# Autodesk Inventor assembly: SingleSpeed_12x64-01
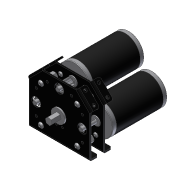
[picture p0: Inventor's stored thumbnail of the model, 180x180]
Saved by Autodesk Inventor 2012 (Build 160160000, 160)
## iProperties
Created: 2013-01-06
Part Number: SingleSpeed_12x64-01
Document SubType Name: Assembly
Designer: JesseK
Mass: 3401.94 g
Surface Area: 2125.02 cm^2
Volume: 1305.71 cm^3
Density: 2.60543 g/cm^3
Translation Standard: STEP AP203
FileName: 217-2745.20121217.STEP
PreProcessor: SolidWorks 2012
PostProcessor: Build: 160, Release: 2012 RTM - Date: Tue 03/01/2011
Sent Units: inch
Uncertainty: 1e-05
Author: JesseK
## Documents named in this file (17)
- Z:\UserData\Documents\Inventor\team1885frc\VEXPro\Gearboxes\SingleSpeed_12x64\SingleSpeed_12x64.iam
- Z:\UserData\Documents\Inventor\team1885frc\VEXPro\Gearboxes\SingleSpeed_12x64\217-2745-001 Rev1.ipt
- Z:\UserData\Documents\Inventor\team1885frc\VEXPro\Gearboxes\SingleSpeed_12x64\217-2000 - CIM Motor.ipt
- Z:\UserData\Documents\Inventor\team1885frc\VEXPro\Gearboxes\SingleSpeed_12x64\217-2731.ipt
- Z:\UserData\Documents\Inventor\team1885frc\VEXPro\Gearboxes\SingleSpeed_12x64\217-2734.ipt
- Z:\UserData\Documents\Inventor\team1885frc\VEXPro\Gearboxes\SingleSpeed_12x64\217-2454-004 Rev1.ipt
- Z:\UserData\Documents\Inventor\team1885frc\VEXPro\Gearboxes\SingleSpeed_12x64\SBS1_SBS1032-0500ZC.ipt
- Z:\UserData\Documents\Inventor\team1885frc\VEXPro\Gearboxes\SingleSpeed_12x64\217-2715-001_64t.ipt
- Z:\UserData\Documents\Inventor\team1885frc\VEXPro\Gearboxes\SingleSpeed_12x64\217-2614-001_12t.ipt
- Z:\UserData\Documents\Inventor\team1885frc\VEXPro\Gearboxes\SingleSpeed_12x64\217-2737 Rev1.ipt
- Z:\UserData\Documents\Inventor\team1885frc\VEXPro\Gearboxes\SingleSpeed_12x64\217-2617-002 Rev1_91780A359.ipt
- Z:\UserData\Documents\Inventor\team1885frc\VEXPro\Gearboxes\SingleSpeed_12x64\SBS1_SBS2520-0500SS.ipt
- Z:\UserData\Documents\Inventor\team1885frc\VEXPro\Gearboxes\SingleSpeed_12x64\217-2614-002_98430A132.ipt
- Z:\UserData\Documents\Inventor\team1885frc\VEXPro\Gearboxes\SingleSpeed_12x64\217-2745-002 Rev1.ipt
- Z:\UserData\Documents\Inventor\team1885frc\VEXPro\Gearboxes\SingleSpeed_12x64\217-2428-005 Rev1.ipt
- Z:\UserData\Documents\Inventor\team1885frc\VEXPro\Gearboxes\SingleSpeed_12x64\SBS1_SBS0832-0500SS.ipt
- SingleSpeed_12x64-01.iam
## Components (41 placed, 15 different names)
1. 217-2745-001 Rev1:1 — Mate:1, Mate:2, Mate:3, Mate:4, Mate:5
2. 217-2745-001 Rev1:2 — Mate:6
3. 217-2000 - CIM Motor:1 — Flush:1, Mate:1
4. 217-2000 - CIM Motor:2 — Flush:1
5. 217-2731:1
6. 217-2734:1
7. 217-2454-004 Rev1:1
8. SBS1_SBS1032-0500ZC:1
9. 217-2715-001_64t:1
10. 217-2614-001_12t:1
11. 217-2737 Rev1:1
12. 217-2617-002 Rev1_91780A359:1
13. SBS1_SBS2520-0500SS:1
14. 217-2617-002 Rev1_91780A359:2
15. 217-2617-002 Rev1_91780A359:3
16. 217-2617-002 Rev1_91780A359:4
17. SBS1_SBS2520-0500SS:2
18. SBS1_SBS2520-0500SS:3
19. SBS1_SBS2520-0500SS:4
20. SBS1_SBS2520-0500SS:5
21. SBS1_SBS2520-0500SS:6
22. SBS1_SBS2520-0500SS:7 — Mate:3, Mate:4
23. SBS1_SBS2520-0500SS:8
24. 217-2614-001_12t:2
25. 217-2614-002_98430A132:1
26. 217-2614-002_98430A132:2
27. 217-2614-002_98430A132:3
28. 217-2614-002_98430A132:4
29. SBS1_SBS1032-0500ZC:2
30. SBS1_SBS1032-0500ZC:3
31. SBS1_SBS1032-0500ZC:4
32. SBS1_SBS1032-0500ZC:5
33. SBS1_SBS1032-0500ZC:6
34. 217-2745-002 Rev1:1
35. 217-2428-005 Rev1:1
36. 217-2428-005 Rev1:2
37. SBS1_SBS0832-0500SS:1
38. SBS1_SBS0832-0500SS:2
39. SBS1_SBS0832-0500SS:3
40. SBS1_SBS0832-0500SS:4
41. 217-2000 - CIM Motor:3 — Mate:2, Mate:5, Mate:6
## Relationships (7: Mate 6, Flush 1)
- Flush:1: 217-2000 - CIM Motor:1 ↔ 217-2000 - CIM Motor:2
- Mate:1: 217-2745-001 Rev1:1 ↔ 217-2000 - CIM Motor:1
- Mate:2: 217-2745-001 Rev1:1 ↔ 217-2000 - CIM Motor:3
- Mate:3: 217-2745-001 Rev1:1 ↔ SBS1_SBS2520-0500SS:7
- Mate:4: 217-2745-001 Rev1:1 ↔ SBS1_SBS2520-0500SS:7
- Mate:5: 217-2745-001 Rev1:1 ↔ 217-2000 - CIM Motor:3
- Mate:6: 217-2745-001 Rev1:2 ↔ 217-2000 - CIM Motor:3
